# Autodesk Inventor assembly: Vertical_Fixation_Set
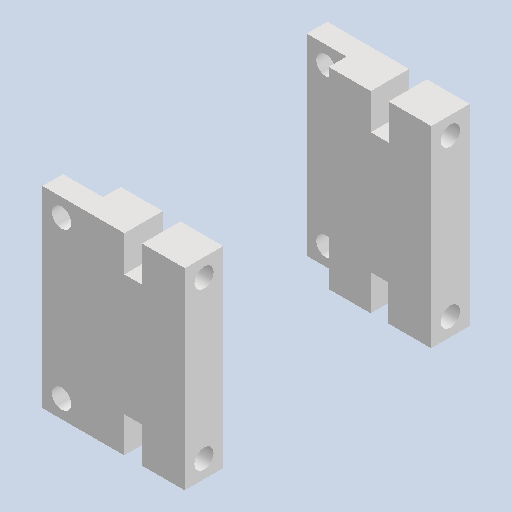
[picture p0: Inventor's stored thumbnail of the model, 512x512]
Saved by Autodesk Inventor 2024.3 (Build 283343000, 343)
## iProperties
Created: 2024-09-06
Part Number: Vertical_Fixation_Set
Document SubType Name: Assembly
Designer: 구지현
Mass: 4.60217 g
Surface Area: 34.4556 cm^2
Volume: 4.60217 cm^3
Density: 1 g/cm^3
Author: 구지현
## Documents named in this file (2)
- C:\Users\구지현\Desktop\HM\Vertical_Fixation_Set.iam
- C:\Users\구지현\Desktop\HM\Vertical_Connector.ipt
## Components (2 placed, 1 different names)
1. Vertical_Connector:1 — 삽입:2, 메이트:1
2. Vertical_Connector:2 — 삽입:2, 메이트:1
## Relationships (2: Insert 1, Mate 1)
- 삽입:2 [Insert] (34.2 mm): Vertical_Connector:1 ↔ Vertical_Connector:2
- 메이트:1 [Mate]: Vertical_Connector:1 ↔ Vertical_Connector:2
